# Autodesk Inventor assembly: 0002_ASS_Ban_lap_ghep_01
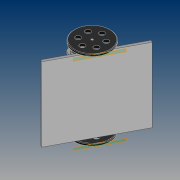
[picture p0: Inventor's stored thumbnail of the model, 180x180]
Saved by Autodesk Inventor 2021 (Build 250183000, 183)
## iProperties
Created: 2024-04-07
Part Number: 0002_ASS_Ban_lap_ghep_01
Document SubType Name: Assembly
Designer: Admin
Author: Admin
## Documents named in this file (3)
- C:\Users\Admin\Desktop\DO_AN_TOT_NGHIEP_2024\Mechanical\Design_in_3D\Version_2\0002_ASS_Ban_lap_ghep_01.iam
- C:\Users\Admin\Desktop\DO_AN_TOT_NGHIEP_2024\Mechanical\Design_in_3D\Version_1\0001_ASS_Hop_so.iam
- C:\Users\Admin\Desktop\DO_AN_TOT_NGHIEP_2024\Mechanical\Design_in_3D\Version_2\01_Tam_de_01.ipt
## Components (3 placed, 2 different names)
1. 0001_ASS_Hop_so:1 [sub-assembly] — Mate:1, Flush:1, Mate:2, Mate:3, Symmetry:1
2. 0001_ASS_Hop_so:2 [sub-assembly] — Mate:1, Flush:1, Mate:2, Mate:4, Symmetry:1
3. 01_Tam_de_01:1 — Mate:3, Mate:4, Mate:5
## Relationships (7: Mate 5, Flush 1, Symmetry 1)
- Mate:1: 0001_ASS_Hop_so:1 ↔ 0001_ASS_Hop_so:2
- Flush:1: 0001_ASS_Hop_so:1 ↔ 0001_ASS_Hop_so:2
- Mate:2 (10 mm): 0001_ASS_Hop_so:1 ↔ 0001_ASS_Hop_so:2
- Mate:3: 0001_ASS_Hop_so:1 ↔ 01_Tam_de_01:1
- Mate:4: 0001_ASS_Hop_so:2 ↔ 01_Tam_de_01:1
- Symmetry:1: 0001_ASS_Hop_so:1 ↔ 0001_ASS_Hop_so:2
- Mate:5: 01_Tam_de_01:1
